# Autodesk Inventor assembly: Fixed_Link_Fixation
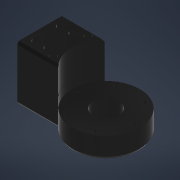
[picture p0: Inventor's stored thumbnail of the model, 180x180]
Saved by Autodesk Inventor 2021 (Build 250183000, 183)
## iProperties
Created: 2025-04-02
Part Number: Fixed_Link_Fixation
Document SubType Name: Assembly
Designer: rocke
Author: rocke
## Documents named in this file (3)
- C:\Users\rocke\Documents\Robot Arm IPT\Fixed Link Fixation\Fixed_Link_Fixation.iam
- C:\Users\rocke\Documents\Robot Arm IPT\Fixed Link Fixation\Fixed_Link_Fixation_Small.ipt
- C:\Users\rocke\Documents\Robot Arm IPT\Fixed Link Fixation\Fixed_Link_Fixation_Large.ipt
## Components (2 placed, 2 different names)
1. Fixed_Link_Fixation_Small:1 — Insert:1
2. Fixed_Link_Fixation_Large:1 — Insert:1
## Relationships (1: Insert 1)
- Insert:1: Fixed_Link_Fixation_Small:1 ↔ Fixed_Link_Fixation_Large:1
